# Autodesk Inventor assembly: IWATA_SCS0608CP3
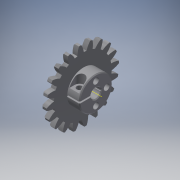
[picture p0: Inventor's stored thumbnail of the model, 180x180]
Saved by Autodesk Inventor 2019 (Build 230136000, 136)
## iProperties
Created: 2020-11-07
Part Number: IWATA_SCS0608CP3
Material: 一般
Document SubType Name: Assembly
Designer: zhept
Author: zhept
## iProperties of the stored document _SCS  0608CP3-part.ipt
Created: 2020-10-06
Part Number: _SCS  0608CP3-part
Material: 一般
Document SubType Name: Modeling
Designer: zhept
Density: 1 g/cm^3
Appearance: 既定
Author: zhept
Revision Number: NONE
## iProperties of the stored document SCS0608CP3.iam
Company: CADENAS
Created: 2020-11-06
Part Number: SCS0608CP3
Material: 一般
Description: STEP AP203
Document SubType Name: Assembly
Designer: zhept
Sending System: PARTsolutions
Title: p:/temp/worker_34/temp/exporttempdir_3780_1137_9iLm4/format_0/SCS0608CP3.stp
Author: License CC BY-ND 4.0
Revision Number: NONE
## Documents named in this file (5)
- **C:\Users\zhept\OneDrive\大学\rrst\足回り2020\IWATA_SCS0608CP3\IWATA_SCS0608CP3.iam*LocalDocs*xI4fxfl4rPmm0e3wt3ngvtfnf0a*_SCS  0608CP3-part.ipt
- **C:\Users\zhept\OneDrive\大学\rrst\足回り2020\IWATA_SCS0608CP3\IWATA_SCS0608CP3.iam*LocalDocs*xMcsss5di1kzqekki1nz5dwaj3c*SCS0608CP3.iam
- C:\Users\zhept\OneDrive\大学\rrst\足回り2020\IWATA_SCS0608CP3\IWATA_SCS0608CP3.iam
- C:\Users\zhept\OneDrive\大学\rrst\足回り2020\KHK_SS220J12On\SS2-20J12_On.ipt
- C:\Users\zhept\OneDrive\大学\rrst\足回り2020\IWATA_SCS0608CP3\SCS0608CP3.stp
## Components (2 placed, 2 different names)
1. SCS0608CP3:1 [sub-assembly] — 挿入:1, 挿入:2, メイト:2
2. SS2-20J12_On:1 — 挿入:1, 挿入:2
## Relationships (4: Insert 2, Mate 2)
- 挿入:1 [Insert]: SCS0608CP3:1 ↔ SS2-20J12_On:1
- 挿入:2 [Insert]: SCS0608CP3:1 ↔ SS2-20J12_On:1
- メイト:2 [Mate]: SCS0608CP3:1
- メイト:3 [Mate]
